# Autodesk Inventor assembly: Wiping unit
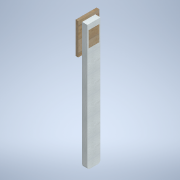
[picture p0: Inventor's stored thumbnail of the model, 180x180]
Saved by Autodesk Inventor 2020 (Build 240168000, 168)
## iProperties
Created: 2021-07-11
Part Number: Wiping unit
Document SubType Name: Assembly
Designer: pc
Author: pc
## Documents named in this file (3)
- C:\Users\pc\Documents\Wiping unit.iam
- C:\Users\pc\Documents\slider.ipt
- C:\Users\pc\Documents\blade1.ipt
## Components (2 placed, 2 different names)
1. slider:1 — Mate:1, Mate:2, Mate:3, Flush:1
2. blade1:1 — Mate:1, Mate:2, Mate:3, Flush:1
## Relationships (4: Mate 3, Flush 1)
- Mate:1: slider:1 ↔ blade1:1
- Mate:2: slider:1 ↔ blade1:1
- Mate:3: slider:1 ↔ blade1:1
- Flush:1: slider:1 ↔ blade1:1
